# Autodesk Inventor assembly: Assembly4
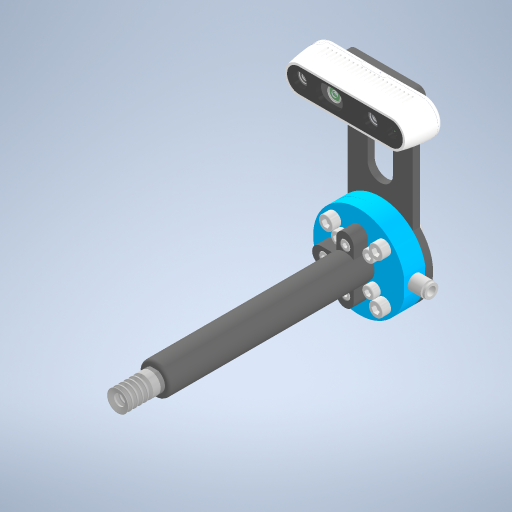
[picture p0: Inventor's stored thumbnail of the model, 512x512]
Saved by Autodesk Inventor 2023 (Build 270158000, 158)
## iProperties
Created: 2022-05-19
Part Number: Assembly4
Document SubType Name: Assembly
Designer: romanp
Author: romanp
## Documents named in this file (12)
- C:\Users\romanp\Downloads\SMC_EE_ZP2-TB15ZJS6-AL12-06\Assembly_SMC_EE.iam
- C:\Users\romanp\Downloads\SMC_EE_ZP2-TB15ZJS6-AL12-06\M4x20.ipt
- C:\Users\romanp\Downloads\SMC_EE_ZP2-TB15ZJS6-AL12-06\M4_nut.ipt
- C:\Users\romanp\Downloads\SMC_EE_ZP2-TB15ZJS6-AL12-06\ZP2-TB15ZJS6-AL12-06.ipt
- C:\Users\romanp\Downloads\SMC_EE_ZP2-TB15ZJS6-AL12-06\IntelRealsense_D435.ipt
- C:\Users\romanp\Downloads\SMC_EE_ZP2-TB15ZJS6-AL12-06\Part_Type_2_Black.ipt
- C:\Users\romanp\Downloads\SMC_EE_ZP2-TB15ZJS6-AL12-06\KQ2H06-00A.ipt
- C:\Users\romanp\Downloads\SMC_EE_ZP2-TB15ZJS6-AL12-06\M5x25.ipt
- C:\Users\romanp\Downloads\SMC_EE_ZP2-TB15ZJS6-AL12-06\M6x25.ipt
- C:\Users\romanp\Downloads\SMC_EE_ZP2-TB15ZJS6-AL12-06\Part_Top_a_Blue.ipt
- C:\Users\romanp\Downloads\SMC_EE_ZP2-TB15ZJS6-AL12-06\Part_Top_b_Blue.ipt
- C:\Users\romanp\Downloads\SMC_EE_ZP2-TB15ZJS6-AL12-06\Part_Bottom_Black.ipt
## Components (21 placed, 11 different names)
1. M4x20:1
2. ZP2-TB15ZJS6-AL12-06:1
3. IntelRealsense_D435:1 — Insert:11, Insert:12
4. Part_Type_2_Black — Insert:11, Insert:12, Insert:13
5. M4x20:2
6. M4x20:3
7. M4_nut:3
8. M4_nut:4
9. M4_nut:5
10. KQ2H06-00A:1
11. M6x25:5 — Insert:15
12. M5x25:5 — Insert:16
13. Part_Top_a_Blue — Insert:13, Insert:14
14. Part_Top_b_Blue — Insert:14, Insert:15, Insert:16, Insert:17, Insert:18, Insert:19, Insert:20, Insert:21, Insert:22, Insert:23
15. M6x25:6 — Insert:18
16. M5x25:6 — Insert:17
17. M6x25:7 — Insert:19
18. M6x25:8 — Insert:20
19. M5x25:7 — Insert:21
20. M5x25:8 — Insert:22
21. Part_Bottom_Black — Insert:23
## Relationships (13: Insert 13)
- Insert:11: IntelRealsense_D435:1 ↔ Part_Type_2_Black
- Insert:12: IntelRealsense_D435:1 ↔ Part_Type_2_Black
- Insert:13: Part_Type_2_Black ↔ Part_Top_a_Blue
- Insert:14: Part_Top_a_Blue ↔ Part_Top_b_Blue
- Insert:15: M6x25:5 ↔ Part_Top_b_Blue
- Insert:16: M5x25:5 ↔ Part_Top_b_Blue
- Insert:17: Part_Top_b_Blue ↔ M5x25:6
- Insert:18: Part_Top_b_Blue ↔ M6x25:6
- Insert:19: Part_Top_b_Blue ↔ M6x25:7
- Insert:20: Part_Top_b_Blue ↔ M6x25:8
- Insert:21: Part_Top_b_Blue ↔ M5x25:7
- Insert:22: Part_Top_b_Blue ↔ M5x25:8
- Insert:23: Part_Top_b_Blue ↔ Part_Bottom_Black
